# Autodesk Inventor assembly: Chassis Assembly
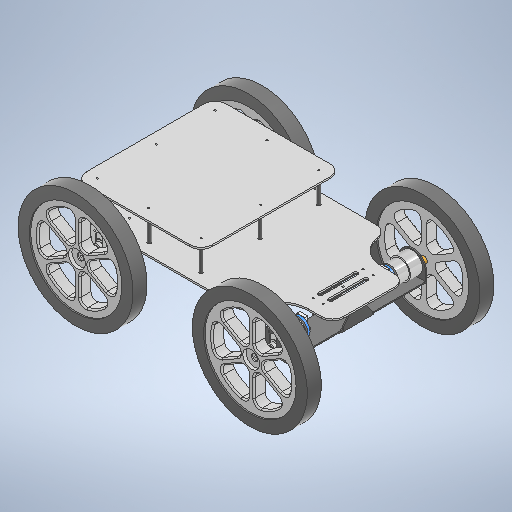
[picture p0: Inventor's stored thumbnail of the model, 512x512]
Saved by Autodesk Inventor 2025.2 (Build 292293000, 293)
## iProperties
Created: 2025-01-16
Part Number: Chassis Assembly
Document SubType Name: Assembly
Designer: Matt Tidd
Author: Matt Tidd
## Documents named in this file (6)
- C:\Users\mtidd\OneDrive\Desktop\H2A\CAD\Chassis_Design\Chassis Assembly.iam
- C:\Users\mtidd\OneDrive\Desktop\H2A\CAD\Motors_and_Wheels\Pendulum Suspension\Pendulum Suspension Assembly.iam
- C:\Users\mtidd\OneDrive\Desktop\H2A\CAD\Chassis_Design\Chassis Bottom Plate.ipt
- C:\Users\mtidd\OneDrive\Desktop\H2A\CAD\Motors_and_Wheels\Wheel Assembly\Motor Wheel Assembly.iam
- C:\Users\mtidd\OneDrive\Desktop\H2A\CAD\Chassis_Design\Support Columns.ipt
- C:\Users\mtidd\OneDrive\Desktop\H2A\CAD\Chassis_Design\Chassis Top Plate.ipt
## Components (13 placed, 5 different names)
1. Pendulum Suspension Assembly:1 [sub-assembly] — Mate:1
2. Chassis Bottom Plate:1 — Mate:1, Mate:2, Mate:3, Mate:4, Mate:5, Mate:17, Mate:18, Mate:19, Mate:20, Mate:21, Mate:22, Mate:23, Mate:24
3. Motor Wheel Assembly:1 [sub-assembly] — Mate:2, Mate:3
4. Motor Wheel Assembly:2 [sub-assembly] — Mate:4, Mate:5
5. Chassis Top Plate:1 — Mate:25
6. Support Columns:1 — Mate:18
7. Support Columns:2 — Mate:20
8. Support Columns:3 — Mate:23
9. Support Columns:4 — Mate:21, Mate:25
10. Support Columns:5 — Mate:22
11. Support Columns:6 — Mate:19
12. Support Columns:7 — Mate:17
13. Support Columns:8 — Mate:24
## Relationships (14: Mate 14)
- Mate:1: Pendulum Suspension Assembly:1 ↔ Chassis Bottom Plate:1
- Mate:2: Chassis Bottom Plate:1 ↔ Motor Wheel Assembly:1
- Mate:3: Chassis Bottom Plate:1 ↔ Motor Wheel Assembly:1
- Mate:4: Chassis Bottom Plate:1 ↔ Motor Wheel Assembly:2
- Mate:5: Chassis Bottom Plate:1 ↔ Motor Wheel Assembly:2
- Mate:17: Chassis Bottom Plate:1 ↔ Support Columns:7
- Mate:18: Chassis Bottom Plate:1 ↔ Support Columns:1
- Mate:19: Chassis Bottom Plate:1 ↔ Support Columns:6
- Mate:20: Chassis Bottom Plate:1 ↔ Support Columns:2
- Mate:21: Chassis Bottom Plate:1 ↔ Support Columns:4
- Mate:22: Chassis Bottom Plate:1 ↔ Support Columns:5
- Mate:23: Chassis Bottom Plate:1 ↔ Support Columns:3
- Mate:24: Chassis Bottom Plate:1 ↔ Support Columns:8
- Mate:25: Chassis Top Plate:1 ↔ Support Columns:4
